# Autodesk Inventor assembly: amazon_universal
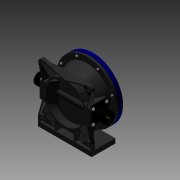
[picture p0: Inventor's stored thumbnail of the model, 180x180]
Saved by Autodesk Inventor 2014 (Build 180170000, 170)
## iProperties
Created: 2013-10-13
Part Number: amazon_universal
Document SubType Name: Assembly
Designer: david
Author: david
## Documents named in this file (10)
- C:\Users\david\Documents\GitHub\CAD\amazon_universal.iam
- C:\Users\david\Documents\GitHub\CAD\SR016_AMUNV_PUMP_BASE.ipt
- C:\Users\david\Documents\GitHub\CAD\RETAINER-RING.ipt
- C:\Users\david\Documents\GitHub\CAD\PIN.ipt
- C:\Users\david\Documents\GitHub\CAD\M-6012_A.iam
- C:\Users\david\Documents\GitHub\CAD\AMAZON_UNIVERSAL_VALVE.ipt
- C:\Users\david\Documents\GitHub\CAD\PORT.ipt
- C:\Users\david\Documents\GitHub\CAD\SCREW-10.ipt
- C:\Users\david\Documents\GitHub\CAD\M-6057.ipt
- C:\Users\david\Documents\GitHub\CAD\bracket.ipt
## Components (26 placed, 9 different names)
1. SR016_AMUNV_PUMP_BASE:1
2. RETAINER-RING:1
3. PIN:2 — Insert:1
4. M-6012_A:1 [sub-assembly] — Rotational:1, Rotational:2, Rotational:3, Insert:1
5. AMAZON_UNIVERSAL_VALVE:1
6. PORT:1
7. PORT:2
8. SCREW-10:1
9. SCREW-10:2
10. SCREW-10:3
11. SCREW-10:4
12. SCREW-10:5
13. SCREW-10:6
14. SCREW-10:7
15. SCREW-10:8
16. SCREW-10:9
17. SCREW-10:10
18. SCREW-10:11
19. SCREW-10:12
20. SCREW-10:13
21. SCREW-10:14
22. SCREW-10:15
23. SCREW-10:16
24. M-6057:1 — Rotational:3
25. bracket:2 — Rotational:1
26. bracket:3 — Rotational:2
## Relationships (4: RevoluteJoint 3, Insert 1)
- Rotational:1 [RevoluteJoint]: M-6012_A:1 ↔ bracket:2
- Rotational:2 [RevoluteJoint]: M-6012_A:1 ↔ bracket:3
- Rotational:3 [RevoluteJoint]: M-6012_A:1 ↔ M-6057:1
- Insert:1: PIN:2 ↔ M-6012_A:1
